# Autodesk Inventor assembly: al_frame
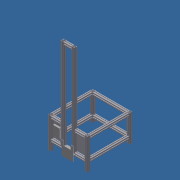
[picture p0: Inventor's stored thumbnail of the model, 180x180]
Saved by Autodesk Inventor 2012 (Build 160160000, 160)
## iProperties
Created: 2012-03-08
Part Number: al_frame
Document SubType Name: Assembly
Designer: esv
Mass: 187059 g
Surface Area: 125343 cm^2
Volume: 160092 cm^3
Density: 1.16845 g/cm^3
Author: esv
## Documents named in this file (12)
- C:\Users\Edward\Documents\masters\CAD\al_frame.iam
- C:\Users\Edward\Documents\masters\CAD\Frame\lower side rail.ipt
- C:\Users\Edward\Documents\masters\CAD\Frame\lower front rail.ipt
- C:\Users\Edward\Documents\masters\CAD\Frame\lower vertical rail.ipt
- C:\Users\Edward\Documents\masters\CAD\Frame\arm rail.ipt
- C:\Users\Edward\Documents\masters\CAD\Frame\front upright.ipt
- C:\Users\Edward\Documents\masters\CAD\Frame\front top side rail.ipt
- C:\Users\Edward\Documents\masters\CAD\Frame\aim rail cross brace.ipt
- C:\Users\Edward\Documents\masters\CAD\LIDAR Power Supply\LIDAR PSU.ipt
- C:\Users\Edward\Documents\masters\CAD\Frame\front right plate.ipt
- C:\Users\Edward\Documents\masters\CAD\Frame\front left plate.ipt
- C:\Users\Edward\Documents\masters\CAD\SICK\LIDAR Bracket.ipt
## Components (20 placed, 11 different names)
1. lower side rail:1 — Flush:9, Flush:12, Flush:14, Flush:76, Mate:108, Flush:84
2. lower side rail:2 — Flush:9, Mate:6, Flush:10, Flush:12, Flush:13, Flush:41, Flush:42, Mate:45, Flush:81
3. lower side rail:3 — Flush:8, Mate:6, Flush:11, Flush:14, Flush:71
4. lower side rail:4 — Flush:8, Flush:10, Flush:11, Flush:13
5. arm rail:1 — Flush:26, Flush:35, Mate:49, Mate:53
6. arm rail:2 — Flush:26, Flush:35, Mate:50, Flush:49, Flush:50, Flush:65, Mate:115
7. front upright:1 — Flush:41, Flush:42, Mate:45, Mate:47, Flush:46, Flush:47, Mate:51, Mate:101, Flush:78
8. front upright:2 — Flush:43, Flush:44, Flush:45, Mate:52, Flush:71, Mate:103, Flush:79
9. lower front rail:3 — Mate:47, Flush:43, Flush:84, Mate:115, Mate:116, Mate:117
10. front top side rail:1 — Flush:46, Flush:47, Mate:50, Mate:51, Flush:55
11. front top side rail:2 — Mate:49, Flush:44, Flush:45, Mate:52, Flush:55
12. aim rail cross brace:1 — Flush:49, Flush:50, Mate:53
13. LIDAR PSU:1 — Flush:65, Tangent:5, Tangent:6
14. lower vertical rail:1 — Flush:69, Flush:70, Flush:74, Flush:75, Mate:100
15. lower vertical rail:2 — Flush:69, Flush:70, Mate:107, Mate:108, Flush:81
16. lower front rail:4 — Flush:72, Flush:73, Flush:74, Flush:75, Mate:100
17. lower front rail:5 — Flush:72, Flush:73, Flush:76, Mate:107
18. front right plate:1 — Mate:101, Flush:78, Flush:80, Tangent:5, Tangent:6
19. front left plate:1 — Mate:103, Flush:79, Flush:80
20. LIDAR Bracket:1 — Mate:116, Mate:117
## Relationships (53: Flush 34, Mate 17, Tangent 2)
- Flush:8: lower side rail:3 ↔ lower side rail:4
- Flush:9: lower side rail:1 ↔ lower side rail:2
- Mate:6 (450.85 mm): lower side rail:2 ↔ lower side rail:3
- Flush:10: lower side rail:2 ↔ lower side rail:4
- Flush:11: lower side rail:3 ↔ lower side rail:4
- Flush:12: lower side rail:1 ↔ lower side rail:2
- Flush:13: lower side rail:2 ↔ lower side rail:4
- Flush:14: lower side rail:1 ↔ lower side rail:3
- Flush:26: arm rail:1 ↔ arm rail:2
- Flush:35: arm rail:1 ↔ arm rail:2
- Flush:40 (-368.3 mm)
- Flush:41: lower side rail:2 ↔ front upright:1
- Flush:42: lower side rail:2 ↔ front upright:1
- Mate:45: lower side rail:2 ↔ front upright:1
- Mate:47: front upright:1 ↔ lower front rail:3
- Flush:43: front upright:2 ↔ lower front rail:3
- Mate:49: arm rail:1 ↔ front top side rail:2
- Flush:44: front upright:2 ↔ front top side rail:2
- Flush:45: front upright:2 ↔ front top side rail:2
- Flush:46: front upright:1 ↔ front top side rail:1
- Flush:47: front upright:1 ↔ front top side rail:1
- Mate:50: arm rail:2 ↔ front top side rail:1
- Mate:51: front upright:1 ↔ front top side rail:1
- Mate:52: front upright:2 ↔ front top side rail:2
- Flush:49: arm rail:2 ↔ aim rail cross brace:1
- Flush:50: arm rail:2 ↔ aim rail cross brace:1
- Mate:53: arm rail:1 ↔ aim rail cross brace:1
- Mate:56
- Flush:55: front top side rail:1 ↔ front top side rail:2
- Flush:65: arm rail:2 ↔ LIDAR PSU:1
- Flush:69: lower vertical rail:1 ↔ lower vertical rail:2
- Flush:70: lower vertical rail:1 ↔ lower vertical rail:2
- Flush:71: lower side rail:3 ↔ front upright:2
- Flush:72: lower front rail:4 ↔ lower front rail:5
- Flush:73: lower front rail:4 ↔ lower front rail:5
- Flush:74: lower vertical rail:1 ↔ lower front rail:4
- Flush:75: lower vertical rail:1 ↔ lower front rail:4
- Mate:100: lower vertical rail:1 ↔ lower front rail:4
- Flush:76: lower side rail:1 ↔ lower front rail:5
- Mate:101: front upright:1 ↔ front right plate:1
- Flush:78: front upright:1 ↔ front right plate:1
- Mate:103: front upright:2 ↔ front left plate:1
- Flush:79: front upright:2 ↔ front left plate:1
- Flush:80: front right plate:1 ↔ front left plate:1
- Tangent:5: LIDAR PSU:1 ↔ front right plate:1
- Tangent:6: LIDAR PSU:1 ↔ front right plate:1
- Mate:107: lower vertical rail:2 ↔ lower front rail:5
- Mate:108: lower side rail:1 ↔ lower vertical rail:2
- Flush:81: lower side rail:2 ↔ lower vertical rail:2
- Flush:84: lower side rail:1 ↔ lower front rail:3
- Mate:115: arm rail:2 ↔ lower front rail:3
- Mate:116: lower front rail:3 ↔ LIDAR Bracket:1
- Mate:117: lower front rail:3 ↔ LIDAR Bracket:1
